# Autodesk Inventor assembly: wheel_assy
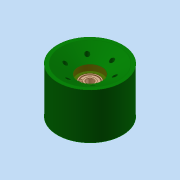
[picture p0: Inventor's stored thumbnail of the model, 180x180]
Saved by Autodesk Inventor 2015 SP1 (Build 190203100, 203)
## iProperties
Created: 2015-06-13
Part Number: wheel_assy
Document SubType Name: Assembly
Designer: YOUR_NAME_HERE
Author: YOUR_NAME_HERE
## Documents named in this file (4)
- C:\Users\Rahul\Electric Skateboard\Electric Skateboard CAD\Imported Components\suspension_assy\wheel_assy_modifiedwheel.iam
- C:\Users\Rahul\Electric Skateboard\Electric Skateboard CAD\Imported Components\suspension_assy\groove_ball_bearing_-_608-z_0.iam
- C:\Users\Rahul\Electric Skateboard\Electric Skateboard CAD\Imported Components\suspension_assy\spacer.ipt
- C:\Users\Rahul\Electric Skateboard\Electric Skateboard CAD\LongboardWheel_modified.ipt
## Components (4 placed, 3 different names)
1. groove_ball_bearing_-_608-z_0:1 [sub-assembly] — Mate:1, Flush:1
2. wheel:1 — Mate:1, Flush:1
3. groove_ball_bearing_-_608-z_0:2 [sub-assembly]
4. spacer:1
## Relationships (2: Mate 1, Flush 1)
- Mate:1: groove_ball_bearing_-_608-z_0:1 ↔ wheel:1
- Flush:1: groove_ball_bearing_-_608-z_0:1 ↔ wheel:1
